# Autodesk Inventor assembly: Тележка для баллона
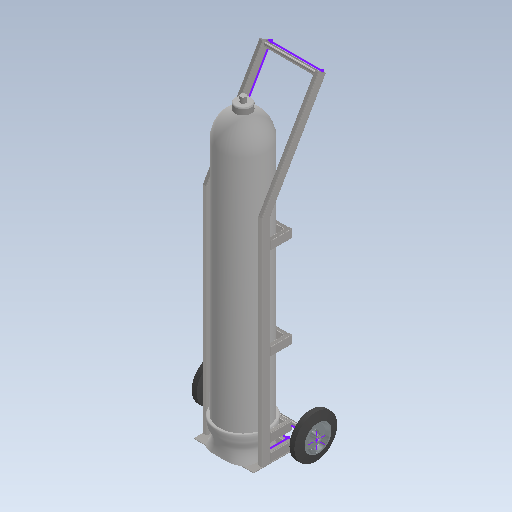
[picture p0: Inventor's stored thumbnail of the model, 512x512]
Saved by Autodesk Inventor 2025.2 (Build 292293000, 293)
## iProperties
Created: 2025-01-20
Part Number: Тележка для баллона
Document SubType Name: Assembly
Designer: neket
_SolveAssemblyDoc: Frame Generator Solve Assembly
_Version: 25.0.0
Author: neket
## Documents named in this file (6)
- C:\Users\neket\OneDrive\Документы\Inventor\Работа\Тележка для баллона.iam
- C:\Users\neket\OneDrive\Документы\Inventor\Работа\Баллон газовый.ipt
- C:\Users\neket\OneDrive\Документы\Inventor\Работа\Каркас тележки.ipt
- C:\Users\neket\OneDrive\Документы\Inventor\Работа\Колесо.ipt
- C:\Users\neket\OneDrive\Документы\Inventor\Работа\Тележка для баллона\Frame\Frame 1737338819388.iam
- C:\Users\neket\OneDrive\Документы\Inventor\Работа\Платформа.ipt
## Components (6 placed, 5 different names)
1. Баллон газовый:1 — Жесткий:1
2. Каркас тележки:1 — Совмещение:1
3. Колесо:1 — Совмещение:3
4. Колесо:2 — Совмещение:2
5. Frame 1737338819388:1 [sub-assembly] — Совмещение:1, Совмещение:2, Совмещение:3, Заподлицо:1
6. Платформа:1 — Заподлицо:1, Жесткий:1
## Relationships (5: Mate 3, Flush 1, WeldJoint 1)
- Совмещение:1 [Mate]: Каркас тележки:1 ↔ Frame 1737338819388:1
- Совмещение:2 [Mate]: Колесо:2 ↔ Frame 1737338819388:1
- Совмещение:3 [Mate]: Колесо:1 ↔ Frame 1737338819388:1
- Заподлицо:1 [Flush]: Frame 1737338819388:1 ↔ Платформа:1
- Жесткий:1 [WeldJoint]: Баллон газовый:1 ↔ Платформа:1
